# Autodesk Inventor assembly: langstroth_10frame
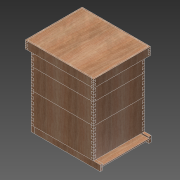
[picture p0: Inventor's stored thumbnail of the model, 180x180]
Saved by Autodesk Inventor 2014 SP1 (Build 180222100, 222)
## iProperties
Created: 2014-02-23
Part Number: langstroth_10frame
Document SubType Name: Assembly
Designer: Chris
Mass: 28565.1 g
Surface Area: 44228.8 cm^2
Volume: 28565.1 cm^3
Density: 1 g/cm^3
Author: Chris
## Documents named in this file (7)
- C:\Users\Chris\Documents\projects\langstroth_plain\langstroth_10frame.iam
- C:\Users\Chris\Documents\projects\langstroth_plain\botton_board\bottom_board.iam
- C:\Users\Chris\Documents\projects\langstroth_plain\deep\deep.iam
- C:\Users\Chris\Documents\projects\langstroth_plain\medium\medium.iam
- C:\Users\Chris\Documents\projects\langstroth_plain\shallow\shallow.iam
- C:\Users\Chris\Documents\projects\langstroth_plain\inner_cover\inner_cover.iam
- C:\Users\Chris\Documents\projects\langstroth_plain\outer_cover\outer_cover.iam
## Components (6 placed, 6 different names)
1. bottom_board:1 [sub-assembly] — Flush:1, Flush:2, Mate:1
2. deep:1 [sub-assembly] — Flush:1, Flush:2, Mate:1, Flush:3, Flush:4, Mate:2
3. medium:1 [sub-assembly] — Flush:3, Flush:4, Mate:2, Flush:5, Mate:3, Flush:6, Flush:7
4. shallow:1 [sub-assembly] — Flush:5, Mate:3, Flush:6, Flush:7, Mate:4, Flush:8, Flush:9
5. inner_cover:1 [sub-assembly] — Mate:4, Flush:8, Flush:9, Mate:5, Mate:6, Mate:7
6. outer_cover:1 [sub-assembly] — Mate:5, Mate:6, Mate:7
## Relationships (16: Flush 9, Mate 7)
- Flush:1: bottom_board:1 ↔ deep:1
- Flush:2: bottom_board:1 ↔ deep:1
- Mate:1: bottom_board:1 ↔ deep:1
- Flush:3: deep:1 ↔ medium:1
- Flush:4: deep:1 ↔ medium:1
- Mate:2: deep:1 ↔ medium:1
- Flush:5: medium:1 ↔ shallow:1
- Mate:3: medium:1 ↔ shallow:1
- Flush:6: medium:1 ↔ shallow:1
- Flush:7: medium:1 ↔ shallow:1
- Mate:4: shallow:1 ↔ inner_cover:1
- Flush:8: shallow:1 ↔ inner_cover:1
- Flush:9: shallow:1 ↔ inner_cover:1
- Mate:5: inner_cover:1 ↔ outer_cover:1
- Mate:6: inner_cover:1 ↔ outer_cover:1
- Mate:7: inner_cover:1 ↔ outer_cover:1
